# Autodesk Inventor assembly: ASY NDM-VOS_powder_hopper
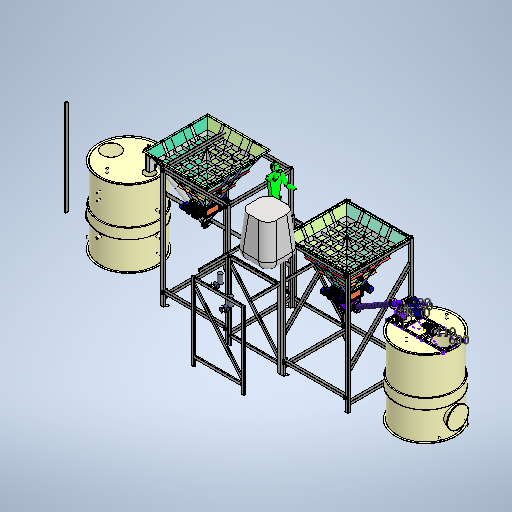
[picture p0: Inventor's stored thumbnail of the model, 512x512]
Saved by Autodesk Inventor 2025.1 (Build 291241020, 241B)
## iProperties
Created: 2024-07-24
Part Number: ASY NDM-VOS_powder_hopper
Document SubType Name: Assembly
Designer: admin
Author: admin
## Documents named in this file (25)
- C:\Users\user\YandexDisk-badmisterfox\домашниий пк\Inventor\NDM-VOS_powder_hopper\ASY NDM-VOS_powder_hopper.iam
- C:\Users\user\YandexDisk-badmisterfox\домашниий пк\Inventor\NDM-VOS_powder_hopper\human 01\ч ASY human dummy 01.iam
- C:\Users\user\YandexDisk-badmisterfox\домашниий пк\Inventor\NDM-VOS_powder_hopper\NDM-VOS dummy3.ipt
- C:\Users\user\YandexDisk-badmisterfox\домашниий пк\Inventor\NDM-VOS_powder_hopper\NDM-VOS dummy FLOOR.ipt
- C:\Users\user\YandexDisk-badmisterfox\домашниий пк\Inventor\NDM-VOS_powder_hopper\NDM-VOS dummy Crane.ipt
- C:\Users\user\YandexDisk-badmisterfox\домашниий пк\Inventor\NDM-VOS_powder_hopper\NDM-VOS dummy upstairse.ipt
- C:\Users\user\YandexDisk-badmisterfox\домашниий пк\Inventor\NDM-VOS_powder_hopper\Workspaces\Workspace\Cone\ASY MSC 100 cone.iam
- C:\Users\user\YandexDisk-badmisterfox\домашниий пк\Inventor\NDM-VOS_powder_hopper\ASY HPR 200  Frame.iam
- C:\Users\user\YandexDisk-badmisterfox\домашниий пк\Inventor\NDM-VOS_powder_hopper\TM06198C pump.ipt
- C:\Users\user\YandexDisk-badmisterfox\домашниий пк\Inventor\NDM-VOS_powder_hopper\ASY_Ступень.iam
- C:\Users\user\YandexDisk-badmisterfox\домашниий пк\Inventor\NDM-VOS_powder_hopper\ASY стойка.iam
- C:\Users\user\YandexDisk-badmisterfox\домашниий пк\Inventor\NDM-VOS_powder_hopper\ISO 4019 - 80x40x2 - 2500.ipt
- C:\Users\user\YandexDisk-badmisterfox\домашниий пк\Inventor\NDM-VOS_powder_hopper\ASY NVPH-400 shredder.iam
- C:\Users\user\YandexDisk-badmisterfox\домашниий пк\Inventor\Content Center Files\en-US\ISO 4775\ISO 4775 - M12.ipt
- C:\Users\user\YandexDisk-badmisterfox\домашниий пк\Inventor\NDM-VOS_powder_hopper\ASY NVPH-300 hopper.iam
- C:\Users\user\YandexDisk-badmisterfox\домашниий пк\Inventor\NDM-VOS_powder_hopper\ASY Augur motor frame 500.iam
- C:\Users\user\YandexDisk-badmisterfox\домашниий пк\Inventor\NDM-VOS_powder_hopper\3d party\motor-reductor NMRV040\motor-reductor NMRV040.iam
- C:\Users\user\YandexDisk-badmisterfox\домашниий пк\Inventor\NDM-VOS_powder_hopper\3d party\Mixer 22.04.24\ASY mixer 3.iam
- C:\Users\user\YandexDisk-badmisterfox\домашниий пк\Inventor\NDM-VOS_powder_hopper\NDM-VOS 777 sredder wall 7.ipt
- C:\Users\user\YandexDisk-badmisterfox\домашниий пк\Inventor\NDM-VOS_powder_hopper\NDM-VOS 778 engine plate.ipt
- C:\Users\user\YandexDisk-badmisterfox\домашниий пк\Inventor\NDM-VOS_powder_hopper\3d party\PCRV071-063SHFA_MS71B5\PCRV071-063SHFA_MS71B5\PCRV071-063SHFA_MS71B5.ipt
- C:\Users\user\YandexDisk-badmisterfox\домашниий пк\Inventor\NDM-VOS_powder_hopper\NDM-VOS 712 flange.ipt
- C:\Users\user\YandexDisk-badmisterfox\домашниий пк\Inventor\NDM-VOS_powder_hopper\NDM-VOS 913 flange bolt.ipt
- C:\Users\user\YandexDisk-badmisterfox\домашниий пк\Inventor\NDM-VOS_powder_hopper\NDM-VOS 715 flange.ipt
- C:\Users\user\YandexDisk-badmisterfox\домашниий пк\Inventor\NDM-VOS_powder_hopper\FL3.6.2  Motor pillar.ipt
## Components (48 placed, 24 different names)
1. NDM-VOS dummy3:2 — Mate:6, Mate:8, Mate:9
2. ч ASY human dummy 01:1 [sub-assembly]
3. NDM-VOS dummy FLOOR:1 — Mate:5, Mate:6, Mate:8, Mate:10, Mate:18
4. NDM-VOS dummy Crane:1 — Mate:10
5. NDM-VOS dummy upstairse:1 — Mate:18, Mate:23
6. ASY MSC 100 CONE:1 [sub-assembly] — Mate:20, Rigid:27, Mate:35, Mate:36
7. ASY HPR 200  Frame:1 [sub-assembly] — Mate:20, Rigid:31, Rigid:32, Mate:35, Mate:36
8. TM06198C pump:1
9. ASY HPR 200  Frame:2 [sub-assembly] — Rigid:33
10. ASY стойка:1 [sub-assembly] — Rigid:5, Rigid:6, Rigid:32, Rigid:33
11. ASY стойка:2 [sub-assembly] — Rigid:4, Rigid:31, Mate:37, Flush:29, Flush:30
12. ASY стойка:3 [sub-assembly] — Rigid:4, Flush:25
13. ISO 4019 - 80x40x2 - 2700:1 — Rigid:5
14. ISO 4019 - 80x40x2 - 2700:2
15. ISO 4019 - 80x40x2 - 2700:3 — Rigid:6, Flush:24, Mate:24, Mate:38, Flush:31
16. ASY MSC 100 CONE:2 [sub-assembly] — Rigid:29
17. TM06198C pump:2
18. ASY NVPH-400 shredder:1 [sub-assembly] — Rigid:27, Mate:31, Mate:32
19. ISO 4775 M12:1 — Mate:31, Mate:32
20. ASY NVPH-300 hopper:1 [sub-assembly] — Rigid:34
21. ASY NVPH-400 shredder:2 [sub-assembly] — Rigid:29, Rigid:30
22. ASY NVPH-300 hopper:2 [sub-assembly] — Rigid:30
23. NDM-VOS dummy3:1 — Mate:5, Mate:9
24. ASY Augur motor frame 500:1 [sub-assembly] — Mate:40, Mate:42, Flush:34, Mate:43, Flush:35, Mate:44, Mate:45, Flush:36
25. motor-reductor NMRV040:1 [sub-assembly] — Rotational:15
26. ASY mixer 3:1 [sub-assembly] — Rotational:15
27. NDM-VOS 112 sredder wall sub:1 — Rigid:34, Rigid:35
28. NDM-VOS 778 engine plate:1 — Rigid:35, Rigid:36, Mate:39, Mate:41
29. PCRV071-063SHFA_MS71B5:1 — Rigid:36
30. NDM-VOS 712 flange:1 — Mate:39, Mate:40, Flush:32, Flush:33
31. NDM-VOS 913 flange bolt:1 — Mate:37, Flush:29, Flush:30
32. NDM-VOS 913 flange bolt:2 — Mate:38, Flush:31
33. NDM-VOS 712 flange:2 — Mate:41, Flush:32, Flush:33
34. NDM-VOS 715 flange:1 — Mate:42, Flush:34
35. FL3.6.2  Motor pillar:1 — Mate:43, Flush:35, Mate:44
36. NDM-VOS 715 flange:2 — Mate:45, Flush:36
37. ASY_Ступень:1 [sub-assembly] — Flush:24, Mate:23, Mate:24, Flush:25
38. ASY_Ступень:2 [sub-assembly]
39. ASY_Ступень:3 [sub-assembly]
40. ASY_Ступень:4 [sub-assembly]
41. ASY_Ступень:5 [sub-assembly]
42. ASY_Ступень:6 [sub-assembly]
43. ASY_Ступень:7 [sub-assembly]
44. ASY_Ступень:8 [sub-assembly]
45. ASY_Ступень:9 [sub-assembly]
46. ASY_Ступень:10 [sub-assembly]
47. ASY_Ступень:11 [sub-assembly]
48. ASY_Ступень:12 [sub-assembly]
## Component patterns: (12 elements, first: ASY_Ступень:1)
## Relationships (54: Mate 26, Flush 14, WeldJoint 13, RevoluteJoint 1)
- Mate:5: NDM-VOS dummy FLOOR:1 ↔ NDM-VOS dummy3:1
- Mate:6: NDM-VOS dummy3:2 ↔ NDM-VOS dummy FLOOR:1
- Mate:8 (1200 mm): NDM-VOS dummy3:2 ↔ NDM-VOS dummy FLOOR:1
- Mate:9 (-1830 mm): NDM-VOS dummy3:2 ↔ NDM-VOS dummy3:1
- Mate:10 (3500 mm): NDM-VOS dummy FLOOR:1 ↔ NDM-VOS dummy Crane:1
- [Mate]: NDM-VOS dummy3:2 ↔ ASY MSC 100 CONE:1
- Mate:18: NDM-VOS dummy FLOOR:1 ↔ NDM-VOS dummy upstairse:1
- [Flush]: ASY HPR 200  Frame:1
- Mate:20: ASY MSC 100 CONE:1 ↔ ASY HPR 200  Frame:1
- Rigid:4 [WeldJoint] (1000 mm): ASY стойка:2 ↔ ASY стойка:3
- Rigid:5 [WeldJoint]: ASY стойка:1 ↔ ISO 4019 - 80x40x2 - 2700:1
- Rigid:6 [WeldJoint]: ASY стойка:1 ↔ ISO 4019 - 80x40x2 - 2700:3
- Flush:24 (182 mm): ISO 4019 - 80x40x2 - 2700:3 ↔ ASY_Ступень:1
- Mate:23: NDM-VOS dummy upstairse:1 ↔ ASY_Ступень:1
- Mate:24: ISO 4019 - 80x40x2 - 2700:3 ↔ ASY_Ступень:1
- Flush:25: ASY стойка:3 ↔ ASY_Ступень:1
- Rigid:27 [WeldJoint]: ASY MSC 100 CONE:1 ↔ ASY NVPH-400 shredder:1
- [WeldJoint]: ASY NVPH-400 shredder:1 ↔ ASY NVPH-300 hopper:1
- [Mate]: ASY NVPH-400 shredder:1 ↔ ASY NVPH-300 hopper:1
- [Flush]: ASY NVPH-400 shredder:1 ↔ ASY NVPH-300 hopper:1
- Mate:31: ASY NVPH-400 shredder:1 ↔ ISO 4775 M12:1
- Mate:32: ASY NVPH-400 shredder:1 ↔ ISO 4775 M12:1
- [Mate]: ASY NVPH-400 shredder:1 ↔ ASY NVPH-300 hopper:1
- Rigid:29 [WeldJoint]: ASY MSC 100 CONE:2 ↔ ASY NVPH-400 shredder:2
- Rigid:30 [WeldJoint]: ASY NVPH-400 shredder:2 ↔ ASY NVPH-300 hopper:2
- [Flush]: NDM-VOS dummy3:1 ↔ ASY Augur motor frame 500:1
- [Mate]: NDM-VOS dummy3:1 ↔ ASY Augur motor frame 500:1
- [Flush]: NDM-VOS dummy3:1 ↔ ASY Augur motor frame 500:1
- Rigid:31 [WeldJoint]: ASY HPR 200  Frame:1 ↔ ASY стойка:2
- Rigid:32 [WeldJoint]: ASY HPR 200  Frame:1 ↔ ASY стойка:1
- Rigid:33 [WeldJoint]: ASY HPR 200  Frame:2 ↔ ASY стойка:1
- Mate:35: ASY MSC 100 CONE:1 ↔ ASY HPR 200  Frame:1
- Mate:36: ASY MSC 100 CONE:1 ↔ ASY HPR 200  Frame:1
- Rotational:15 [RevoluteJoint]: motor-reductor NMRV040:1 ↔ ASY mixer 3:1
- Mate:37: ASY стойка:2 ↔ NDM-VOS 913 flange bolt:1
- Flush:29: ASY стойка:2 ↔ NDM-VOS 913 flange bolt:1
- Flush:30: ASY стойка:2 ↔ NDM-VOS 913 flange bolt:1
- Mate:38: ISO 4019 - 80x40x2 - 2700:3 ↔ NDM-VOS 913 flange bolt:2
- Flush:31: ISO 4019 - 80x40x2 - 2700:3 ↔ NDM-VOS 913 flange bolt:2
- Rigid:34 [WeldJoint]: ASY NVPH-300 hopper:1 ↔ NDM-VOS 112 sredder wall sub:1
- Rigid:35 [WeldJoint]: NDM-VOS 112 sredder wall sub:1 ↔ NDM-VOS 778 engine plate:1
- Rigid:36 [WeldJoint]: NDM-VOS 778 engine plate:1 ↔ PCRV071-063SHFA_MS71B5:1
- Mate:39: NDM-VOS 778 engine plate:1 ↔ NDM-VOS 712 flange:1
- Mate:40 (380 mm): ASY Augur motor frame 500:1 ↔ NDM-VOS 712 flange:1
- Mate:41: NDM-VOS 778 engine plate:1 ↔ NDM-VOS 712 flange:2
- Flush:32: NDM-VOS 712 flange:1 ↔ NDM-VOS 712 flange:2
- Flush:33: NDM-VOS 712 flange:1 ↔ NDM-VOS 712 flange:2
- Mate:42: ASY Augur motor frame 500:1 ↔ NDM-VOS 715 flange:1
- Flush:34: ASY Augur motor frame 500:1 ↔ NDM-VOS 715 flange:1
- Mate:43: ASY Augur motor frame 500:1 ↔ FL3.6.2  Motor pillar:1
- Flush:35: ASY Augur motor frame 500:1 ↔ FL3.6.2  Motor pillar:1
- Mate:44: ASY Augur motor frame 500:1 ↔ FL3.6.2  Motor pillar:1
- Mate:45: ASY Augur motor frame 500:1 ↔ NDM-VOS 715 flange:2
- Flush:36: ASY Augur motor frame 500:1 ↔ NDM-VOS 715 flange:2
